# Autodesk Inventor assembly: jigAndRunnerAssembly
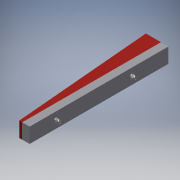
[picture p0: Inventor's stored thumbnail of the model, 180x180]
Saved by Autodesk Inventor 2019.1 (Build 231200000, 200)
## iProperties
Created: 2018-08-02
Part Number: jigAndRunnerAssembly
Document SubType Name: Assembly
Designer: steele
Author: steele
## Documents named in this file (5)
- C:\git\CAD-Development\robSteele\HouseProjects\TableSaw\jigAndRunnerAssembly.iam
- C:\git\CAD-Development\robSteele\HouseProjects\TableSaw\tableSawRunner.ipt
- C:\git\CAD-Development\robSteele\HouseProjects\TableSaw\jigForRipCuts.ipt
- C:\git\CAD-Development\robSteele\HouseProjects\TableSaw\jigAndRunnerAssembly\Design Accelerator\Bolted Connection1.iam
- C:\git\CAD-Development\robSteele\HouseProjects\TableSaw\jigAndRunnerAssembly\Design Accelerator\Bolted Connection2.iam
## Components (4 placed, 3 different names)
1. tableSawRunner:1 — Insert:1, Insert:2
2. jigForRipCuts:1 — Insert:1, Insert:2, Mate:1, Mate:2, Mate:3, Mate:4
3. Bolted Connection:1 [sub-assembly] — Mate:1, Mate:2
4. Bolted Connection:2 [sub-assembly] — Mate:3, Mate:4
## Relationships (6: Mate 4, Insert 2)
- Insert:1: tableSawRunner:1 ↔ jigForRipCuts:1
- Insert:2: tableSawRunner:1 ↔ jigForRipCuts:1
- Mate:1: jigForRipCuts:1 ↔ Bolted Connection:1
- Mate:2: jigForRipCuts:1 ↔ Bolted Connection:1
- Mate:3: jigForRipCuts:1 ↔ Bolted Connection:2
- Mate:4: jigForRipCuts:1 ↔ Bolted Connection:2
